# Autodesk Inventor assembly: 知能ロボコンギアボックス改
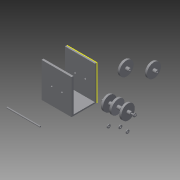
[picture p0: Inventor's stored thumbnail of the model, 180x180]
Saved by Autodesk Inventor 2013 (Build 170138000, 138)
## iProperties
Created: 2014-06-02
Part Number: 知能ロボコンギアボックス改
Document SubType Name: Assembly
Designer: horumo136
Author: horumo136
## Documents named in this file (5)
- C:\Users\horumo136\Documents\知能ロボコンギアボックス改.iam
- C:\Users\horumo136\Documents\知能ロボコンギアボックス１.ipt
- C:\Users\horumo136\Documents\知能ロボコンアルミギア１０３Ｃ.ipt
- C:\Users\horumo136\Documents\知能ロボコンシャフト.ipt
- C:\Users\horumo136\Documents\知能ロボコンスペーサ―.ipt
## Components (15 placed, 4 different names)
1. 知能ロボコンギアボックス１:1
2. 知能ロボコンアルミギア１０３Ｃ:1 — メイト:1
3. 知能ロボコンアルミギア１０３Ｃ:2
4. 知能ロボコンアルミギア１０３Ｃ:3 — メイト:5
5. 知能ロボコンアルミギア１０３Ｃ:4
6. 知能ロボコンアルミギア１０３Ｃ:5 — メイト:4
7. 知能ロボコンシャフト:1
8. 知能ロボコンシャフト:2 — メイト:1, メイト:2, メイト:3, メイト:4, メイト:5, メイト:6, メイト:7
9. 知能ロボコンスペーサ―:1 — メイト:3
10. 知能ロボコンスペーサ―:2 — メイト:2
11. 知能ロボコンスペーサ―:3 — メイト:6
12. 知能ロボコンスペーサ―:4
13. 知能ロボコンスペーサ―:5
14. 知能ロボコンスペーサ―:6
15. 知能ロボコンスペーサ―:7 — メイト:7
## Relationships (7: Mate 7)
- メイト:1 [Mate]: 知能ロボコンアルミギア１０３Ｃ:1 ↔ 知能ロボコンシャフト:2
- メイト:2 [Mate]: 知能ロボコンシャフト:2 ↔ 知能ロボコンスペーサ―:2
- メイト:3 [Mate]: 知能ロボコンシャフト:2 ↔ 知能ロボコンスペーサ―:1
- メイト:4 [Mate]: 知能ロボコンアルミギア１０３Ｃ:5 ↔ 知能ロボコンシャフト:2
- メイト:5 [Mate]: 知能ロボコンアルミギア１０３Ｃ:3 ↔ 知能ロボコンシャフト:2
- メイト:6 [Mate]: 知能ロボコンシャフト:2 ↔ 知能ロボコンスペーサ―:3
- メイト:7 [Mate]: 知能ロボコンシャフト:2 ↔ 知能ロボコンスペーサ―:7
